# Autodesk Inventor assembly: NeedleValueTurner
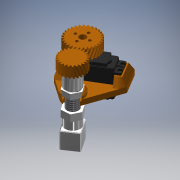
[picture p0: Inventor's stored thumbnail of the model, 180x180]
Saved by Autodesk Inventor 2017.3 (Build 213256000, 256)
## iProperties
Created: 2019-11-14
Part Number: NeedleValueTurner
Document SubType Name: Assembly
Designer: guberti
Author: guberti
## Documents named in this file (5)
- C:\Users\guberti\Documents\2019 - 2020 School Year\Inventor\NeedleValueTurner.iam
- C:\Users\guberti\Documents\2019 - 2020 School Year\Inventor\NeedleValveServoMount.ipt
- C:\Users\guberti\Documents\2019 - 2020 School Year\Inventor\NeedleValveCAD.ipt
- C:\Users\guberti\Documents\2019 - 2020 School Year\Inventor\NeedleValueTurner\Design Accelerator\Spur Gears2.iam
- C:\Users\guberti\Documents\2019 - 2020 School Year\Inventor\Tetrix Servo with Horn.ipt
## Components (4 placed, 4 different names)
1. NeedleValveServoMount:1 — Mate:3, Mate:4, Mate:5, Mate:11, Mate:12, Mate:13
2. NeedleValveCAD:1 — Mate:3, Mate:4, Mate:5, Mate:8, Mate:10
3. Spur Gears:1 [sub-assembly] — Mate:8, Mate:10, Mate:14
4. Tetrix Servo with Horn:1 — Mate:11, Mate:12, Mate:13, Mate:14
## Relationships (9: Mate 9)
- Mate:3: NeedleValveServoMount:1 ↔ NeedleValveCAD:1
- Mate:4: NeedleValveServoMount:1 ↔ NeedleValveCAD:1
- Mate:5: NeedleValveServoMount:1 ↔ NeedleValveCAD:1
- Mate:8: NeedleValveCAD:1 ↔ Spur Gears:1
- Mate:10: NeedleValveCAD:1 ↔ Spur Gears:1
- Mate:11: NeedleValveServoMount:1 ↔ Tetrix Servo with Horn:1
- Mate:12: NeedleValveServoMount:1 ↔ Tetrix Servo with Horn:1
- Mate:13: NeedleValveServoMount:1 ↔ Tetrix Servo with Horn:1
- Mate:14: Spur Gears:1 ↔ Tetrix Servo with Horn:1
